# Autodesk Inventor assembly: WheelGuardsAssembled
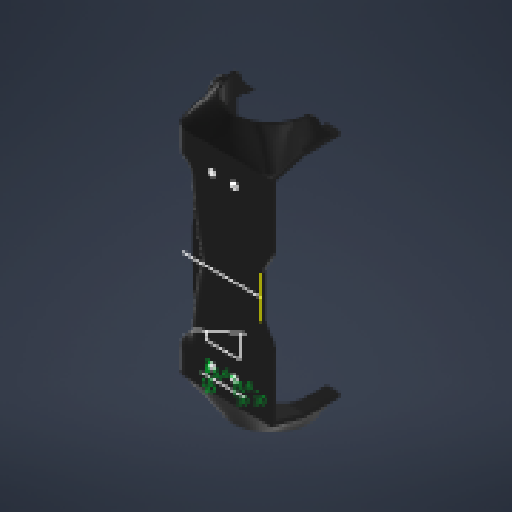
[picture p0: Inventor's stored thumbnail of the model, 512x512]
Saved by Autodesk Inventor 2023 (Build 270158000, 158)
## iProperties
Created: 2023-10-08
Part Number: WheelGuardsAssembled
Document SubType Name: Assembly
Designer: khrip
Author: khrip
## Documents named in this file (3)
- C:\GitHub\Botik\WheelGuardsAssembled.iam
- C:\GitHub\Botik\WheelGuards.ipt
- C:\GitHub\Botik\WheelExtenshions.ipt
## Components (3 placed, 2 different names)
1. WheelGuards:1 — Совмещение:1, Совмещение:2, Заподлицо:1, Совмещение:3, Совмещение:4, Заподлицо:2
2. WheelExtenshions:1 — Совмещение:1, Совмещение:2, Заподлицо:1
3. WheelExtenshions:2 — Совмещение:3, Совмещение:4, Заподлицо:2
## Relationships (6: Mate 4, Flush 2)
- Совмещение:1 [Mate]: WheelGuards:1 ↔ WheelExtenshions:1
- Совмещение:2 [Mate]: WheelGuards:1 ↔ WheelExtenshions:1
- Заподлицо:1 [Flush]: WheelGuards:1 ↔ WheelExtenshions:1
- Совмещение:3 [Mate]: WheelGuards:1 ↔ WheelExtenshions:2
- Совмещение:4 [Mate]: WheelGuards:1 ↔ WheelExtenshions:2
- Заподлицо:2 [Flush]: WheelGuards:1 ↔ WheelExtenshions:2
